# Autodesk Inventor assembly: FullField-ver2-1111-2021
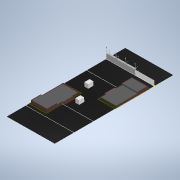
[picture p0: Inventor's stored thumbnail of the model, 180x180]
Saved by Autodesk Inventor 2021 (Build 250183000, 183)
## iProperties
Created: 2021-02-23
Part Number: FullField-ver2-1111-2021
Document SubType Name: Assembly
Designer: CMurray
Author: CMurray
## Documents named in this file (8)
- F:\PHRC CADD 2021\2021 Game Design Challenge\Full Field\Final Assembly\FullField-ver2-1111-2021.iam
- F:\PHRC CADD 2021\2021 Game Design Challenge\Full Field\Parts\FieldFloor-ver1-1111-2021.ipt
- F:\PHRC CADD 2021\2021 Game Design Challenge\Full Field\Parts\Tape\Tape.ipt
- F:\PHRC CADD 2021\2021 Game Design Challenge\Full Field\Parts\Tape\RedAllianceTape-ver1-1111-2021.ipt
- F:\PHRC CADD 2021\2021 Game Design Challenge\Full Field\Parts\Tape\BlueAllianceTape-ver1-1111-2021.ipt
- F:\PHRC CADD 2021\2021 Game Design Challenge\Main Ship\ShipDesign-ver4-1111-2021.ipt
- F:\PHRC CADD 2021\2021 Game Design Challenge\Misc\MockRobot-ver1-1111-2021.ipt
- F:\PHRC CADD 2021\2021 Game Design Challenge\Player Station\Assemblies\DriverStation-ver1-1111-2021.iam
## Components (15 placed, 7 different names)
1. FieldFloor-ver1-1111-2021:1 — Flush:1, Flush:2, Mate:1, Mate:3, Mate:10, Flush:10, Mate:14, Flush:12, Mate:16, Mate:20, Flush:13
2. FieldFloor-ver1-1111-2021:2 — Flush:1, Flush:2, Mate:1, Mate:2, Flush:3, Flush:4, Flush:5, Flush:6, Mate:4, Flush:7, Mate:6, Flush:8, Mate:8, Flush:9, Mate:12, Flush:11, Mate:17, Mate:18, Mate:19
3. ShipDesign-ver4-1111-2021:1 — Mate:16
4. ShipDesign-ver4-1111-2021:2 — Mate:17
5. MockRobot-ver1-1111-2021:1 — Mate:18
6. MockRobot-ver1-1111-2021:2 — Mate:19
7. DriverStation-ver1-1111-2021:1 [sub-assembly] — Mate:20, Flush:13, Mate:21
8. Tape:1 — Mate:2, Flush:3, Flush:4, Mate:5, Mate:9, Mate:11
9. Tape:2 — Mate:3, Flush:5, Flush:6, Mate:7, Mate:13, Mate:15, Mate:21
10. Tape:3 — Mate:4, Flush:7, Mate:5
11. Tape:4 — Mate:6, Flush:8, Mate:7
12. RedAllianceTape-ver1-1111-2021:1 — Mate:8, Flush:9, Mate:9
13. RedAllianceTape-ver1-1111-2021:2 — Mate:10, Flush:10, Mate:11
14. BlueAllianceTape-ver1-1111-2021:1 — Mate:12, Flush:11, Mate:13
15. BlueAllianceTape-ver1-1111-2021:2 — Mate:14, Flush:12, Mate:15
## Relationships (34: Mate 21, Flush 13)
- Flush:1: FieldFloor-ver1-1111-2021:1 ↔ FieldFloor-ver1-1111-2021:2
- Flush:2: FieldFloor-ver1-1111-2021:1 ↔ FieldFloor-ver1-1111-2021:2
- Mate:1: FieldFloor-ver1-1111-2021:1 ↔ FieldFloor-ver1-1111-2021:2
- Mate:2: FieldFloor-ver1-1111-2021:2 ↔ Tape:1
- Flush:3: FieldFloor-ver1-1111-2021:2 ↔ Tape:1
- Flush:4 (3606.8 mm): FieldFloor-ver1-1111-2021:2 ↔ Tape:1
- Mate:3: FieldFloor-ver1-1111-2021:1 ↔ Tape:2
- Flush:5: FieldFloor-ver1-1111-2021:2 ↔ Tape:2
- Flush:6 (3606.8 mm): FieldFloor-ver1-1111-2021:2 ↔ Tape:2
- Mate:4: FieldFloor-ver1-1111-2021:2 ↔ Tape:3
- Flush:7: FieldFloor-ver1-1111-2021:2 ↔ Tape:3
- Mate:5 (3657.6 mm): Tape:1 ↔ Tape:3
- Mate:6: FieldFloor-ver1-1111-2021:2 ↔ Tape:4
- Flush:8: FieldFloor-ver1-1111-2021:2 ↔ Tape:4
- Mate:7 (3657.6 mm): Tape:2 ↔ Tape:4
- Mate:8: FieldFloor-ver1-1111-2021:2 ↔ RedAllianceTape-ver1-1111-2021:1
- Flush:9: FieldFloor-ver1-1111-2021:2 ↔ RedAllianceTape-ver1-1111-2021:1
- Mate:9: Tape:1 ↔ RedAllianceTape-ver1-1111-2021:1
- Mate:10: FieldFloor-ver1-1111-2021:1 ↔ RedAllianceTape-ver1-1111-2021:2
- Flush:10: FieldFloor-ver1-1111-2021:1 ↔ RedAllianceTape-ver1-1111-2021:2
- Mate:11: Tape:1 ↔ RedAllianceTape-ver1-1111-2021:2
- Mate:12: FieldFloor-ver1-1111-2021:2 ↔ BlueAllianceTape-ver1-1111-2021:1
- Flush:11: FieldFloor-ver1-1111-2021:2 ↔ BlueAllianceTape-ver1-1111-2021:1
- Mate:13: Tape:2 ↔ BlueAllianceTape-ver1-1111-2021:1
- Mate:14: FieldFloor-ver1-1111-2021:1 ↔ BlueAllianceTape-ver1-1111-2021:2
- Flush:12: FieldFloor-ver1-1111-2021:1 ↔ BlueAllianceTape-ver1-1111-2021:2
- Mate:15: Tape:2 ↔ BlueAllianceTape-ver1-1111-2021:2
- Mate:16: FieldFloor-ver1-1111-2021:1 ↔ ShipDesign-ver4-1111-2021:1
- Mate:17: FieldFloor-ver1-1111-2021:2 ↔ ShipDesign-ver4-1111-2021:2
- Mate:18: FieldFloor-ver1-1111-2021:2 ↔ MockRobot-ver1-1111-2021:1
- Mate:19: FieldFloor-ver1-1111-2021:2 ↔ MockRobot-ver1-1111-2021:2
- Mate:20: FieldFloor-ver1-1111-2021:1 ↔ DriverStation-ver1-1111-2021:1
- Flush:13: FieldFloor-ver1-1111-2021:1 ↔ DriverStation-ver1-1111-2021:1
- Mate:21: DriverStation-ver1-1111-2021:1 ↔ Tape:2
